# Autodesk Inventor assembly: P1704_E001
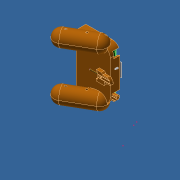
[picture p0: Inventor's stored thumbnail of the model, 180x180]
Saved by Autodesk Inventor 2019 (Build 230136000, 136)
## iProperties
Created: 2019-04-29
Part Number: P1704_E001
Material: Générique
Document SubType Name: Assembly
Designer: Joan.MAILLARD
Author: Joan.MAILLARD
## Documents named in this file (13)
- P:\projet_manette\manette\06_Dessins\2019\Manette universelle\P1704_E001.iam
- P:\projet_manette\manette\06_Dessins\2019\Manette universelle\P1704_004_mainDroiteExterieur.ipt
- P:\projet_manette\manette\06_Dessins\2019\Manette universelle\P1704_005_mainGaucheExterieur.ipt
- P:\projet_manette\manette\06_Dessins\2019\Manette universelle\P1704_001_basManette.ipt
- P:\projet_manette\manette\06_Dessins\2019\Manette universelle\P1704_006_gachette.ipt
- P:\projet_manette\manette\06_Dessins\2019\Manette universelle\P1704_007_guideRessort.ipt
- P:\projet_manette\manette\06_Dessins\2019\Manette universelle\P1704_002_mainDroiteInterieur.ipt
- P:\projet_manette\manette\06_Dessins\2019\Manette universelle\P1704_003_mainGaucheInterieur.ipt
- P:\projet_manette\manette\06_Dessins\2019\Manette universelle\P1704_009_slider.ipt
- P:\projet_manette\manette\06_Dessins\2019\Manette universelle\pcb_boutons.ipt
- P:\projet_manette\manette\06_Dessins\2019\Manette universelle\pcb_central.ipt
- P:\projet_manette\manette\06_Dessins\2019\Manette universelle\pcb_intelligence.ipt
- P:\projet_manette\manette\06_Dessins\2019\Manette universelle\display.ipt
## Components (16 placed, 12 different names)
1. P1704_004_mainDroiteExterieur:1 — Rotation:7, Rotation:8, Placage:14
2. P1704_005_mainGaucheExterieur:1 — Rotation:9, Rotation:10, Placage:12
3. P1704_001_basManette:1 — Placage:1, Placage:2, Placage:3, Placage:7, Placage:8, Placage:9, Placage:10, Placage:11, Placage:12, Placage:13, Placage:14, Placage:15
4. P1704_006_gachette:1 — Rotation:2, Glissière:4
5. P1704_006_gachette:2 — Rotation:1, Glissière:3
6. P1704_007_guideRessort:1 — Rotation:1
7. P1704_007_guideRessort:2 — Rotation:2
8. P1704_002_mainDroiteInterieur:1 — Rotation:7, Rotation:8, Placage:13
9. P1704_003_mainGaucheInterieur:1 — Rotation:9, Rotation:10, Placage:11
10. P1704_009_slider:1 — Glissière:3
11. P1704_009_slider:2 — Glissière:4
12. manette_2019_boutons.kicad_pcb_Contour:1 — Placage:6, Placage:7
13. manette_2019_boutons.kicad_pcb_Contour:2 — Placage:5, Placage:8
14. Manette_2019_PCB_Central.kicad_pcb_Contour:1 — Placage:4, Placage:9, Placage:10, Affleurement:1
15. manette_2019.kicad_pcb_Contour:1 — Placage:1, Placage:2, Placage:3, Placage:4, Placage:5, Placage:6
16. display:1 — Affleurement:1, Placage:15
## Relationships (24: Mate 15, RevoluteJoint 6, TranslationJoint 2, Flush 1)
- Rotation:1 [RevoluteJoint] (4.5 mm): P1704_006_gachette:2 ↔ P1704_007_guideRessort:1
- Rotation:2 [RevoluteJoint] (4.5 mm): P1704_006_gachette:1 ↔ P1704_007_guideRessort:2
- Rotation:7 [RevoluteJoint]: P1704_004_mainDroiteExterieur:1 ↔ P1704_002_mainDroiteInterieur:1
- Rotation:8 [RevoluteJoint]: P1704_004_mainDroiteExterieur:1 ↔ P1704_002_mainDroiteInterieur:1
- Rotation:9 [RevoluteJoint]: P1704_005_mainGaucheExterieur:1 ↔ P1704_003_mainGaucheInterieur:1
- Rotation:10 [RevoluteJoint]: P1704_005_mainGaucheExterieur:1 ↔ P1704_003_mainGaucheInterieur:1
- Glissière:3 [TranslationJoint]: P1704_006_gachette:2 ↔ P1704_009_slider:1
- Glissière:4 [TranslationJoint]: P1704_006_gachette:1 ↔ P1704_009_slider:2
- Placage:1 [Mate]: P1704_001_basManette:1 ↔ manette_2019.kicad_pcb_Contour:1
- Placage:2 [Mate]: P1704_001_basManette:1 ↔ manette_2019.kicad_pcb_Contour:1
- Placage:3 [Mate]: P1704_001_basManette:1 ↔ manette_2019.kicad_pcb_Contour:1
- Placage:4 [Mate] (8 mm): Manette_2019_PCB_Central.kicad_pcb_Contour:1 ↔ manette_2019.kicad_pcb_Contour:1
- Placage:5 [Mate] (8 mm): manette_2019_boutons.kicad_pcb_Contour:2 ↔ manette_2019.kicad_pcb_Contour:1
- Placage:6 [Mate] (8 mm): manette_2019_boutons.kicad_pcb_Contour:1 ↔ manette_2019.kicad_pcb_Contour:1
- Placage:7 [Mate] (8 mm): P1704_001_basManette:1 ↔ manette_2019_boutons.kicad_pcb_Contour:1
- Placage:8 [Mate] (8 mm): P1704_001_basManette:1 ↔ manette_2019_boutons.kicad_pcb_Contour:2
- Placage:9 [Mate] (50 mm): P1704_001_basManette:1 ↔ Manette_2019_PCB_Central.kicad_pcb_Contour:1
- Placage:10 [Mate] (57.5 mm): P1704_001_basManette:1 ↔ Manette_2019_PCB_Central.kicad_pcb_Contour:1
- Placage:11 [Mate]: P1704_001_basManette:1 ↔ P1704_003_mainGaucheInterieur:1
- Placage:12 [Mate]: P1704_005_mainGaucheExterieur:1 ↔ P1704_001_basManette:1
- Placage:13 [Mate]: P1704_001_basManette:1 ↔ P1704_002_mainDroiteInterieur:1
- Placage:14 [Mate]: P1704_004_mainDroiteExterieur:1 ↔ P1704_001_basManette:1
- Affleurement:1 [Flush] (-8 mm): Manette_2019_PCB_Central.kicad_pcb_Contour:1 ↔ display:1
- Placage:15 [Mate] (53.375 mm): P1704_001_basManette:1 ↔ display:1
